# Autodesk Inventor assembly: Assembled
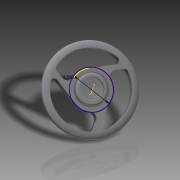
[picture p0: Inventor's stored thumbnail of the model, 180x180]
Saved by Autodesk Inventor 2018 (Build 220112000, 112)
## iProperties
Created: 2017-12-13
Part Number: Assembled
Document SubType Name: Assembly
Designer: Rus
Author: Rus
## Documents named in this file (4)
- E:\Libraries\Documents\3D Models\Spinners and Tops\Circles\Assembled.iam
- E:\Libraries\Documents\3D Models\Spinners and Tops\Caps 8mm\Square Rounded Caps\608-bearing.ipt
- E:\Libraries\Documents\3D Models\Spinners and Tops\Caps 8mm\Square Rounded Caps\Caps 8mm Square Rounded Caps Female.ipt
- E:\Libraries\Documents\3D Models\Spinners and Tops\Circles\Spinner 1.ipt
## Components (4 placed, 3 different names)
1. 608-bearing:1 — Insert:1, Insert:2
2. Caps 8mm Square Rounded Caps Female:1 — Mate:1, Tangent:1, Mate:2, Insert:2, Angle:1
3. Caps 8mm Square Rounded Caps Female:2 — Mate:1, Tangent:1, Mate:2
4. Spinner 1:1 — Insert:1, Angle:1
## Relationships (6: Insert 2, Mate 2, Tangent 1, Angle 1)
- Insert:1: 608-bearing:1 ↔ Spinner 1:1
- Mate:1: Caps 8mm Square Rounded Caps Female:1 ↔ Caps 8mm Square Rounded Caps Female:2
- Tangent:1: Caps 8mm Square Rounded Caps Female:1 ↔ Caps 8mm Square Rounded Caps Female:2
- Mate:2: Caps 8mm Square Rounded Caps Female:1 ↔ Caps 8mm Square Rounded Caps Female:2
- Insert:2: 608-bearing:1 ↔ Caps 8mm Square Rounded Caps Female:1
- Angle:1 (0 deg): Caps 8mm Square Rounded Caps Female:1 ↔ Spinner 1:1
